# Autodesk Inventor assembly: Superstructure-Mount
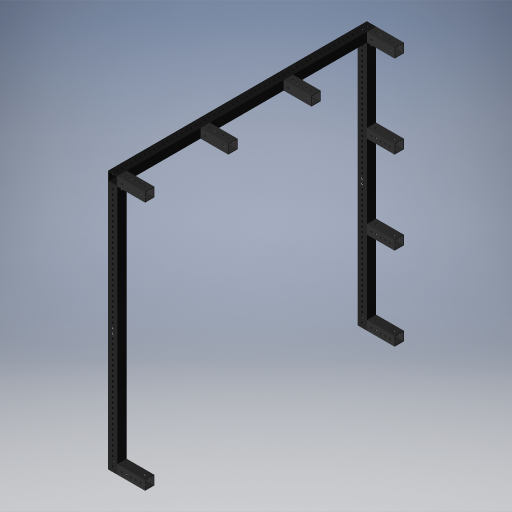
[picture p0: Inventor's stored thumbnail of the model, 512x512]
Saved by Autodesk Inventor 2024.2 (Build 282272000, 272)
## iProperties
Created: 2024-02-11
Part Number: Superstructure-Mount
Document SubType Name: Assembly
Designer: rohan
Author: rohan
## Documents named in this file (4)
- C:\Users\rohan\OneDrive - Hillsborough County Public Schools\Robotics\FIRST-Robotics-Competition\Crescendo\Minotaur-Crescendo-Robot\Structure\Aluminum-Extrusions\Superstructure-Mount.iam
- C:\Users\rohan\OneDrive - Hillsborough County Public Schools\Robotics\FIRST-Robotics-Competition\Crescendo\Minotaur-Crescendo-Robot\Structure\Aluminum-Extrusions\2024-100-009-Structure-Front-Rail.ipt
- C:\Users\rohan\OneDrive - Hillsborough County Public Schools\Robotics\FIRST-Robotics-Competition\Crescendo\Minotaur-Crescendo-Robot\Structure\Aluminum-Extrusions\2024-100-008-Structure-Standoffs.ipt
- C:\Users\rohan\OneDrive - Hillsborough County Public Schools\Robotics\FIRST-Robotics-Competition\Crescendo\Minotaur-Crescendo-Robot\Structure\Aluminum-Extrusions\2024-100-009-Structure-Side-Rail.ipt
## Components (11 placed, 3 different names)
1. 2024-100-009-Structure-Front-Rail:1 — Mate:1, Flush:1, Flush:2, Mate:2, Flush:3, Flush:4, Mate:3, Mate:4, Flush:5, Flush:6, Mate:7, Flush:7, Flush:8, Mate:8, Flush:9, Flush:10
2. 2024-100-008-Structure-Standoffs:1 — Mate:2, Flush:3, Flush:4, Mate:5
3. 2024-100-008-Structure-Standoffs:2 — Mate:1, Flush:1, Flush:2, Mate:6, Flush:15, Mate:14
4. 2024-100-008-Structure-Standoffs:3 — Mate:3, Flush:5, Mate:5
5. 2024-100-008-Structure-Standoffs:4 — Mate:4, Flush:6, Mate:6
6. 2024-100-009-Structure-Side-Rail:1 — Mate:7, Flush:7, Flush:8, Mate:10, Flush:13, Flush:14, Mate:11, Mate:12
7. 2024-100-009-Structure-Side-Rail:2 — Mate:8, Flush:9, Flush:10, Mate:9, Flush:11, Flush:12
8. 2024-100-008-Structure-Standoffs:5 — Mate:10, Flush:13, Flush:14, Flush:16, Mate:13
9. 2024-100-008-Structure-Standoffs:6 — Mate:9, Flush:11, Flush:12
10. 2024-100-008-Structure-Standoffs:7 — Mate:12, Flush:15, Mate:14
11. 2024-100-008-Structure-Standoffs:8 — Mate:11, Flush:16, Mate:13
## Relationships (30: Flush 16, Mate 14)
- Mate:1: 2024-100-009-Structure-Front-Rail:1 ↔ 2024-100-008-Structure-Standoffs:2
- Flush:1: 2024-100-009-Structure-Front-Rail:1 ↔ 2024-100-008-Structure-Standoffs:2
- Flush:2: 2024-100-009-Structure-Front-Rail:1 ↔ 2024-100-008-Structure-Standoffs:2
- Mate:2: 2024-100-009-Structure-Front-Rail:1 ↔ 2024-100-008-Structure-Standoffs:1
- Flush:3: 2024-100-009-Structure-Front-Rail:1 ↔ 2024-100-008-Structure-Standoffs:1
- Flush:4: 2024-100-009-Structure-Front-Rail:1 ↔ 2024-100-008-Structure-Standoffs:1
- Mate:3: 2024-100-009-Structure-Front-Rail:1 ↔ 2024-100-008-Structure-Standoffs:3
- Mate:4: 2024-100-009-Structure-Front-Rail:1 ↔ 2024-100-008-Structure-Standoffs:4
- Flush:5: 2024-100-009-Structure-Front-Rail:1 ↔ 2024-100-008-Structure-Standoffs:3
- Flush:6: 2024-100-009-Structure-Front-Rail:1 ↔ 2024-100-008-Structure-Standoffs:4
- Mate:5 (203.2 mm): 2024-100-008-Structure-Standoffs:1 ↔ 2024-100-008-Structure-Standoffs:3
- Mate:6 (203.2 mm): 2024-100-008-Structure-Standoffs:2 ↔ 2024-100-008-Structure-Standoffs:4
- Mate:7: 2024-100-009-Structure-Front-Rail:1 ↔ 2024-100-009-Structure-Side-Rail:1
- Flush:7: 2024-100-009-Structure-Front-Rail:1 ↔ 2024-100-009-Structure-Side-Rail:1
- Flush:8: 2024-100-009-Structure-Front-Rail:1 ↔ 2024-100-009-Structure-Side-Rail:1
- Mate:8: 2024-100-009-Structure-Front-Rail:1 ↔ 2024-100-009-Structure-Side-Rail:2
- Flush:9: 2024-100-009-Structure-Front-Rail:1 ↔ 2024-100-009-Structure-Side-Rail:2
- Flush:10: 2024-100-009-Structure-Front-Rail:1 ↔ 2024-100-009-Structure-Side-Rail:2
- Mate:9: 2024-100-009-Structure-Side-Rail:2 ↔ 2024-100-008-Structure-Standoffs:6
- Flush:11: 2024-100-009-Structure-Side-Rail:2 ↔ 2024-100-008-Structure-Standoffs:6
- Flush:12: 2024-100-009-Structure-Side-Rail:2 ↔ 2024-100-008-Structure-Standoffs:6
- Mate:10: 2024-100-009-Structure-Side-Rail:1 ↔ 2024-100-008-Structure-Standoffs:5
- Flush:13: 2024-100-009-Structure-Side-Rail:1 ↔ 2024-100-008-Structure-Standoffs:5
- Flush:14: 2024-100-009-Structure-Side-Rail:1 ↔ 2024-100-008-Structure-Standoffs:5
- Mate:11: 2024-100-009-Structure-Side-Rail:1 ↔ 2024-100-008-Structure-Standoffs:8
- Mate:12: 2024-100-009-Structure-Side-Rail:1 ↔ 2024-100-008-Structure-Standoffs:7
- Flush:15: 2024-100-008-Structure-Standoffs:2 ↔ 2024-100-008-Structure-Standoffs:7
- Flush:16: 2024-100-008-Structure-Standoffs:5 ↔ 2024-100-008-Structure-Standoffs:8
- Mate:13 (203.2 mm): 2024-100-008-Structure-Standoffs:5 ↔ 2024-100-008-Structure-Standoffs:8
- Mate:14 (203.2 mm): 2024-100-008-Structure-Standoffs:2 ↔ 2024-100-008-Structure-Standoffs:7
